# Autodesk Inventor assembly: Assembly1
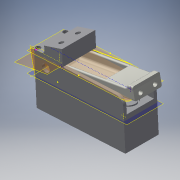
[picture p0: Inventor's stored thumbnail of the model, 180x180]
Saved by Autodesk Inventor 2019 (Build 230136000, 136)
## iProperties
Created: 2021-01-21
Part Number: Assembly1
Material: Genérico
Document SubType Name: Assembly
Designer: Juan M. Casillas
Author: Juan M. Casillas
## Documents named in this file (7)
- K:\3DPrinting\3DModels\shifter\Assembly1.iam
- K:\3DPrinting\3DModels\shifter\microswitch.ipt
- K:\3DPrinting\3DModels\shifter\base_plate.ipt
- K:\3DPrinting\3DModels\shifter\lever.ipt
- K:\3DPrinting\3DModels\shifter\plate.ipt
- K:\3DPrinting\3DModels\shifter\cap.ipt
- K:\3DPrinting\3DModels\shifter\rearcap.ipt
## Components (6 placed, 6 different names)
1. plate:1
2. microswitch:1 — Flush:2
3. base_plate:1 — Flush:2, Flush:3, Mate:1, Mate:2, Rotational:2, Flush:4, Flush:5, Flush:6, Flush:7
4. lever:1 — Mate:1, Mate:2, Rotational:2
5. cap:1 — Flush:4, Flush:5
6. rearcap:1 — Flush:6, Flush:7
## Relationships (9: Flush 6, Mate 2, RevoluteJoint 1)
- Flush:2: microswitch:1 ↔ base_plate:1
- Flush:3 (0.1 mm): base_plate:1
- Mate:1: base_plate:1 ↔ lever:1
- Mate:2: base_plate:1 ↔ lever:1
- Rotational:2 [RevoluteJoint]: base_plate:1 ↔ lever:1
- Flush:4: base_plate:1 ↔ cap:1
- Flush:5: base_plate:1 ↔ cap:1
- Flush:6: base_plate:1 ↔ rearcap:1
- Flush:7: base_plate:1 ↔ rearcap:1
